# Autodesk Inventor assembly: 3-6V DC Gearbox Electromotor
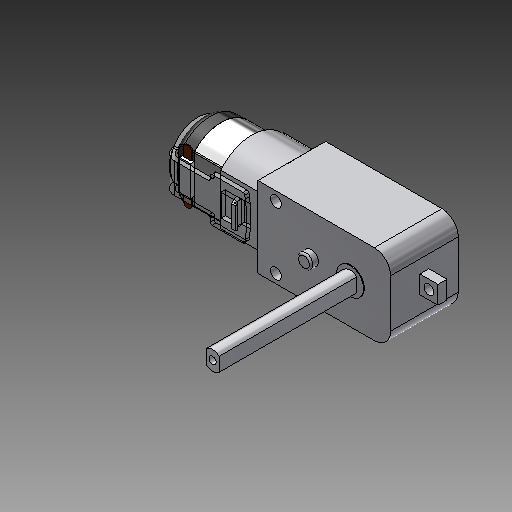
[picture p0: Inventor's stored thumbnail of the model, 512x512]
Saved by Autodesk Inventor 2019 (Build 230136000, 136)
## iProperties
Created: 2020-10-25
Part Number: 3-6V DC Gearbox Electromotor
Document SubType Name: Assembly
Designer: Niels
Author: Niels
## Documents named in this file (4)
- C:\Users\saeva\OneDrive\Desktop\motor\3-6V DC Gearbox Electromotor.iam
- C:\Users\saeva\OneDrive\Desktop\motor\DC 3-6V Gearbox Motor.ipt
- C:\Users\saeva\OneDrive\Desktop\motor\3V DC Electromotor.ipt
- C:\Users\saeva\OneDrive\Desktop\motor\Part3 - Gearbox.ipt
## Components (3 placed, 3 different names)
1. DC 3-6V Gearbox Motor:1 — Insert:1, Mate:1, Flush:1
2. 3V DC Electromotor:1 — Insert:1, Mate:1
3. Part3 - Gearbox:1 — Flush:2
## Relationships (4: Flush 2, Insert 1, Mate 1)
- Insert:1: DC 3-6V Gearbox Motor:1 ↔ 3V DC Electromotor:1
- Mate:1 (0.15 mm): DC 3-6V Gearbox Motor:1 ↔ 3V DC Electromotor:1
- Flush:1 (-3 mm): DC 3-6V Gearbox Motor:1
- Flush:2: Part3 - Gearbox:1
